# Autodesk Inventor assembly: ensamblaje-2sillas
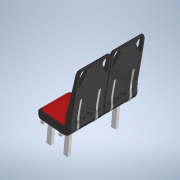
[picture p0: Inventor's stored thumbnail of the model, 180x180]
Saved by Autodesk Inventor 2021 (Build 250183000, 183)
## iProperties
Created: 2022-05-07
Part Number: ensamblaje-2sillas
Document SubType Name: Assembly
Designer: luzve
Author: luzve
## Documents named in this file (5)
- C:\Users\luzve\Documents\Git\SediaAutomatica\Draft\new-bus-seat-1.snapshot.1\ensamblaje-2sillas.iam
- C:\Users\luzve\Documents\Git\SediaAutomatica\Draft\new-bus-seat-1.snapshot.1\ensamblaje-silla.iam
- C:\Users\luzve\Documents\Git\SediaAutomatica\Draft\new-bus-seat-1.snapshot.1\perfil-cuadrado.ipt
- C:\Users\luzve\Documents\Git\SediaAutomatica\Draft\new-bus-seat-1.snapshot.1\lamina1.ipt
- C:\Users\luzve\Documents\Git\SediaAutomatica\Draft\new-bus-seat-1.snapshot.1\leg.ipt
## Components (10 placed, 4 different names)
1. ensamblaje-silla:1 [sub-assembly] — Rígido:1, Rígido:2
2. ensamblaje-silla:2 [sub-assembly] — De rotación:1
3. perfil-cuadrado:1 — Rígido:1, De rotación:1, Rígido:3, Rígido:4
4. perfil-cuadrado:2 — Rígido:2
5. lamina1:1 — Rígido:3, Rígido:7, Rígido:8
6. lamina1:2 — Rígido:4, Rígido:5, Rígido:6
7. leg:1 — Rígido:5
8. leg:2 — Rígido:7
9. leg:3 — Rígido:8
10. leg:4 — Rígido:6
## Relationships (9: WeldJoint 8, RevoluteJoint 1)
- Rígido:1 [WeldJoint]: ensamblaje-silla:1 ↔ perfil-cuadrado:1
- De rotación:1 [RevoluteJoint]: ensamblaje-silla:2 ↔ perfil-cuadrado:1
- Rígido:2 [WeldJoint]: ensamblaje-silla:1 ↔ perfil-cuadrado:2
- Rígido:3 [WeldJoint]: perfil-cuadrado:1 ↔ lamina1:1
- Rígido:4 [WeldJoint]: perfil-cuadrado:1 ↔ lamina1:2
- Rígido:5 [WeldJoint]: lamina1:2 ↔ leg:1
- Rígido:6 [WeldJoint]: lamina1:2 ↔ leg:4
- Rígido:7 [WeldJoint]: lamina1:1 ↔ leg:2
- Rígido:8 [WeldJoint]: lamina1:1 ↔ leg:3
